# Autodesk Inventor assembly: intake second stage
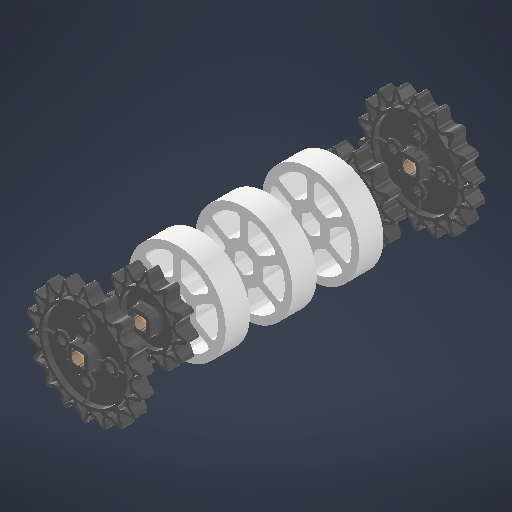
[picture p0: Inventor's stored thumbnail of the model, 512x512]
Saved by Autodesk Inventor 2025.2 (Build 292293000, 293)
## iProperties
Created: 2025-12-04
Part Number: intake second stage
Document SubType Name: Assembly
Designer: cloudy
Author: cloudy
## Documents named in this file (6)
- C:\Users\cloudy\Documents\GitHub\aura-cad\15\intake second stage.iam
- C:\Users\cloudy\Documents\GitHub\aura-cad\!lib\Motion\Sprockets\9P Sprocket\9P 12T Sprocket, No Insert.iam
- C:\Users\cloudy\Documents\GitHub\aura-cad\!lib\Motion\Sprockets\9P Sprocket.iam
- C:\Users\cloudy\Documents\GitHub\aura-cad\!lib\Motion\Wheels\Flex Wheels\2.000 Flex Wheel\2.000 30A .500.ipt
- C:\Users\cloudy\Documents\GitHub\aura-cad\!lib\Motion\Wheels\Flex Wheels\2.000 Flex Wheel.ipt
- C:\Users\cloudy\Documents\GitHub\aura-cad\!lib\Motion\Sprockets\9P Sprocket\9P 18T Sprocket, No Insert.iam
## Components (7 placed, 3 different names)
1. 9P 18T Sprocket, No Insert:1 [sub-assembly] — Insert:1
2. 9P 12T Sprocket, No Insert:2 [sub-assembly] — Insert:1, Insert:2
3. 9P 12T Sprocket, No Insert:3 [sub-assembly] — Insert:5, Insert:6
4. 9P 18T Sprocket, No Insert:4 [sub-assembly] — Insert:6
5. 2.000 30A .500:1 — Insert:2, Insert:3
6. 2.000 30A .500:2 — Insert:3, Insert:4
7. 2.000 30A .500:3 — Insert:4, Insert:5
## Relationships (6: Insert 6)
- Insert:1 (19.05 mm): 9P 18T Sprocket, No Insert:1 ↔ 9P 12T Sprocket, No Insert:2
- Insert:2 (6.35 mm): 9P 12T Sprocket, No Insert:2 ↔ 2.000 30A .500:1
- Insert:3 (22.225 mm): 2.000 30A .500:1 ↔ 2.000 30A .500:2
- Insert:4 (22.225 mm): 2.000 30A .500:2 ↔ 2.000 30A .500:3
- Insert:5 (6.35 mm): 9P 12T Sprocket, No Insert:3 ↔ 2.000 30A .500:3
- Insert:6 (19.05 mm): 9P 12T Sprocket, No Insert:3 ↔ 9P 18T Sprocket, No Insert:4
